# Autodesk Inventor assembly: steadier_grabber
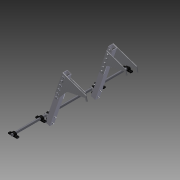
[picture p0: Inventor's stored thumbnail of the model, 180x180]
Saved by Autodesk Inventor 2011 (Build 150239000, 239)
## iProperties
Created: 2013-01-19
Part Number: steadier_grabber
Document SubType Name: Assembly
Designer: Christopher
Author: Christopher
## Documents named in this file (5)
- F:\Users\Christopher\Documents\GitHub\2013CAD\2013 robot\forklift\Pneumatics and frame grabbers\steadier_grabber.iam
- F:\Users\Christopher\Documents\GitHub\2013CAD\2013 robot\forklift\Pneumatics and frame grabbers\right_grabber.iam
- F:\Users\Christopher\Documents\GitHub\2013CAD\2013 robot\forklift\Pneumatics and frame grabbers\left_grabber.iam
- F:\Users\Christopher\Documents\GitHub\2013CAD\2013 robot\forklift\frame parts\0.5unkeyedaxle_26.ipt
- F:\Users\Christopher\Documents\GitHub\2013CAD\2013 robot\forklift\Misc parts\.5inch_side_bearing.ipt
## Components (7 placed, 4 different names)
1. right_grabber:1 [sub-assembly] — Insert:5, Flush:4
2. left_grabber:1 [sub-assembly] — Insert:6, Flush:4
3. 0.5unkeyedaxle_26:1 — Insert:1, Insert:2, Insert:3, Insert:4, Insert:5, Insert:6
4. .5inch_side_bearing:1 — Insert:1, Flush:2
5. .5inch_side_bearing:2 — Insert:2, Flush:1, Flush:2
6. .5inch_side_bearing:3 — Insert:3, Flush:3
7. .5inch_side_bearing:4 — Insert:4, Flush:1, Flush:3
## Relationships (10: Insert 6, Flush 4)
- Insert:1 (6.35 mm): 0.5unkeyedaxle_26:1 ↔ .5inch_side_bearing:1
- Insert:2 (158.75 mm): 0.5unkeyedaxle_26:1 ↔ .5inch_side_bearing:2
- Insert:3 (6.35 mm): 0.5unkeyedaxle_26:1 ↔ .5inch_side_bearing:3
- Insert:4 (158.75 mm): 0.5unkeyedaxle_26:1 ↔ .5inch_side_bearing:4
- Flush:1: .5inch_side_bearing:2 ↔ .5inch_side_bearing:4
- Flush:2: .5inch_side_bearing:1 ↔ .5inch_side_bearing:2
- Flush:3: .5inch_side_bearing:3 ↔ .5inch_side_bearing:4
- Insert:5 (190.5 mm): right_grabber:1 ↔ 0.5unkeyedaxle_26:1
- Insert:6 (190.5 mm): left_grabber:1 ↔ 0.5unkeyedaxle_26:1
- Flush:4: right_grabber:1 ↔ left_grabber:1
